# Autodesk Inventor assembly: tip_3_n_ass
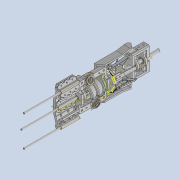
[picture p0: Inventor's stored thumbnail of the model, 180x180]
Saved by Autodesk Inventor 2020 (Build 240168000, 168)
## iProperties
Created: 2021-10-06
Part Number: tip_3_n_ass
Document SubType Name: Assembly
Designer: Shuang Peng
Author: Shuang Peng
## Documents named in this file (11)
- D:\projects-3\torque fb tip\hardware\tip_3\tip_3_n_ass.iam
- D:\projects-3\torque fb tip\hardware\tip_3\roller_n_1.ipt
- D:\projects-3\torque fb tip\hardware\tip_3\bearing_hh_1.ipt
- D:\projects-3\torque fb tip\hardware\tip_3\bearing_3_6_2.ipt
- D:\projects-3\torque fb tip\hardware\tip_3\pin3_40.ipt
- D:\projects-3\torque fb tip\hardware\tip_3\end_shell_n_1.ipt
- D:\projects-3\torque fb tip\hardware\tip_3\c_roller_1.ipt
- D:\projects-3\torque fb tip\hardware\compact_ma_tmp\tip_hl_ass_1.iam
- D:\projects-3\torque fb tip\hardware\tip_3\x_shell_2.ipt
- D:\projects-3\torque fb tip\hardware\tip_3\bl_tube_ass_2.iam
- D:\projects-3\torque fb tip\hardware\tip_3\ext_pin_shell_1.ipt
## Components (23 placed, 10 different names)
1. roller_n_1:1 — Insert:1, Insert:2, Insert:5
2. roller_n_1:2 — Insert:1, Insert:2, Insert:6, Flush:3
3. bearing_hh_1:1 — Insert:3, Flush:1, Flush:2
4. bearing_hh_1:2 — Insert:4, Flush:1, Insert:8
5. bearing_3_6_2:1 — Insert:4, Insert:6
6. bearing_3_6_2:2 — Insert:3, Insert:5, Insert:7
7. pin3_40:1 — Insert:7, Insert:13, Insert:25
8. end_shell_n_1:1 — Flush:2, Insert:8, Flush:3, Insert:10, Insert:12, Flush:4, Insert:14, Insert:22, Flush:6, Insert:23, Insert:24
9. c_roller_1:1 — Insert:9
10. bearing_3_6_2:3 — Insert:9, Insert:10
11. c_roller_1:2
12. bearing_3_6_2:4 — Insert:12
13. tip_hl_ass_1:1 [sub-assembly] — Insert:13
14. x_shell_2:1 — Flush:4, Insert:14, Insert:17, Insert:18, Insert:19, Insert:20, Insert:22
15. bearing_hh_1:3 — Insert:19, Insert:20
16. bearing_3_6_2:5
17. bearing_hh_1:4 — Insert:17, Insert:18
18. bearing_3_6_2:6 — Insert:21
19. pin3_40:2 — Insert:21
20. bl_tube_ass_2:1 [sub-assembly] — Insert:25, Angle:1
21. ext_pin_shell_1:1 — Flush:6, Insert:23, Insert:24, Angle:1, Insert:26, Insert:27, Insert:28, Insert:29
22. bl_tube_ass_2:2 [sub-assembly] — Insert:26, Insert:27
23. bl_tube_ass_2:3 [sub-assembly] — Insert:28, Insert:29
## Relationships (35: Insert 29, Flush 5, Angle 1)
- Insert:1: roller_n_1:1 ↔ roller_n_1:2
- Insert:2: roller_n_1:1 ↔ roller_n_1:2
- Insert:3: bearing_hh_1:1 ↔ bearing_3_6_2:2
- Insert:4: bearing_hh_1:2 ↔ bearing_3_6_2:1
- Insert:5: roller_n_1:1 ↔ bearing_3_6_2:2
- Insert:6: roller_n_1:2 ↔ bearing_3_6_2:1
- Flush:1: bearing_hh_1:1 ↔ bearing_hh_1:2
- Insert:7 (-3 mm): bearing_3_6_2:2 ↔ pin3_40:1
- Flush:2: bearing_hh_1:1 ↔ end_shell_n_1:1
- Insert:8: bearing_hh_1:2 ↔ end_shell_n_1:1
- Flush:3: roller_n_1:2 ↔ end_shell_n_1:1
- Insert:9: c_roller_1:1 ↔ bearing_3_6_2:3
- Insert:10: end_shell_n_1:1 ↔ bearing_3_6_2:3
- [Insert]: c_roller_1:2 ↔ bearing_3_6_2:4
- Insert:12: end_shell_n_1:1 ↔ bearing_3_6_2:4
- Insert:13 (-8 mm): pin3_40:1 ↔ tip_hl_ass_1:1
- Flush:4: end_shell_n_1:1 ↔ x_shell_2:1
- Insert:14: end_shell_n_1:1 ↔ x_shell_2:1
- [Insert]: bearing_hh_1:3 ↔ bearing_3_6_2:5
- [Insert]: bearing_hh_1:4 ↔ bearing_3_6_2:6
- Insert:17: x_shell_2:1 ↔ bearing_hh_1:4
- Insert:18: x_shell_2:1 ↔ bearing_hh_1:4
- Insert:19: x_shell_2:1 ↔ bearing_hh_1:3
- Insert:20: x_shell_2:1 ↔ bearing_hh_1:3
- Insert:21 (-12 mm): bearing_3_6_2:6 ↔ pin3_40:2
- Insert:22: end_shell_n_1:1 ↔ x_shell_2:1
- Flush:6: end_shell_n_1:1 ↔ ext_pin_shell_1:1
- Insert:23: end_shell_n_1:1 ↔ ext_pin_shell_1:1
- Insert:24: end_shell_n_1:1 ↔ ext_pin_shell_1:1
- Insert:25 (1.5 mm): pin3_40:1 ↔ bl_tube_ass_2:1
- Angle:1 (0 deg): bl_tube_ass_2:1 ↔ ext_pin_shell_1:1
- Insert:26: ext_pin_shell_1:1 ↔ bl_tube_ass_2:2
- Insert:27: ext_pin_shell_1:1 ↔ bl_tube_ass_2:2
- Insert:28: ext_pin_shell_1:1 ↔ bl_tube_ass_2:3
- Insert:29: ext_pin_shell_1:1 ↔ bl_tube_ass_2:3
## Named parameters: d13_d11 = 0 mm, d19_d2 = 0 mm, d20_d2 = 0 mm
